# Autodesk Inventor assembly: Drive
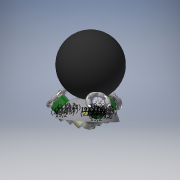
[picture p0: Inventor's stored thumbnail of the model, 180x180]
Saved by Autodesk Inventor 2018.3 (Build 223284000, 284)
## iProperties
Created: 2018-06-30
Part Number: Drive
Material: Generisch
Document SubType Name: Assembly
Designer: JochenAlt
Author: JochenAlt
## Documents named in this file (3)
- D:\Projects\FlowerPot\CAD\Drive.iam
- D:\Projects\FlowerPot\CAD\DriveChain.iam
- D:\Projects\FlowerPot\CAD\Sphere.ipt
## Components (4 placed, 2 different names)
1. Antriebsstrang:1 [sub-assembly] — Passend:1, Passend:3, Passend:5, Tangential:1
2. Antriebsstrang:2 [sub-assembly] — Passend:2, Passend:4
3. Antriebsstrang:3 [sub-assembly] — Passend:1, Passend:2, Passend:3, Passend:4
4. Sphere:1 — Passend:5, Tangential:1
## Relationships (6: Mate 5, Tangent 1)
- Passend:1 [Mate]: Antriebsstrang:1 ↔ Antriebsstrang:3
- Passend:2 [Mate]: Antriebsstrang:2 ↔ Antriebsstrang:3
- Passend:3 [Mate]: Antriebsstrang:1 ↔ Antriebsstrang:3
- Passend:4 [Mate]: Antriebsstrang:2 ↔ Antriebsstrang:3
- Passend:5 [Mate]: Antriebsstrang:1 ↔ Sphere:1
- Tangential:1: Antriebsstrang:1 ↔ Sphere:1
